# Autodesk Inventor assembly: Prueba_ensamble inercia
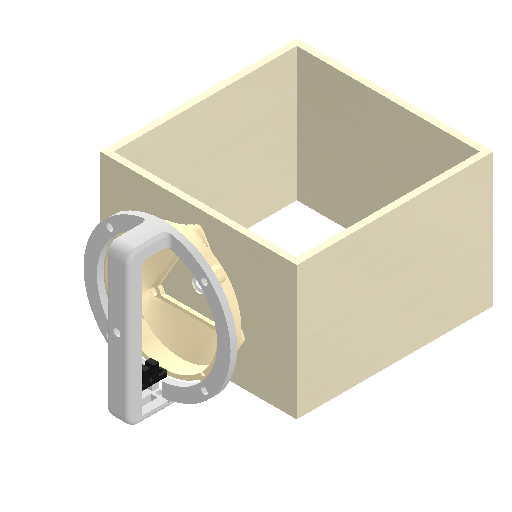
[picture p0: Inventor's stored thumbnail of the model, 512x512]
Saved by Autodesk Inventor 2025.2 (Build 292293000, 293)
## iProperties
Created: 2025-05-05
Part Number: Prueba_ensamble inercia
Document SubType Name: Assembly
Designer: nicoa
Author: nicoa
## Documents named in this file (6)
- C:\Users\nicoa\Documents\FLUSS\Tunel_fluss\Ensamble inercia\Prueba_ensamble inercia.iam
- C:\Users\nicoa\Documents\FLUSS\Tunel_fluss\Ensamble inercia\Seccion_tunel.ipt
- C:\Users\nicoa\Documents\FLUSS\Tunel_fluss\Ensamble inercia\soporte motor.ipt
- C:\Users\nicoa\Documents\FLUSS\Tunel_fluss\Ensamble inercia\Eje_econder.ipt
- C:\Users\nicoa\Documents\FLUSS\Tunel_fluss\Ensamble inercia\Sensor.ipt
- C:\Users\nicoa\Documents\FLUSS\Tunel_fluss\Ensamble inercia\Soporte.ipt
## Components (5 placed, 5 different names)
1. Seccion_tunel:1 — Mate:1, Rotational:1
2. soporte motor:1 — Mate:1, Rotational:1, Mate:2, Mate:3
3. Eje_econder:1
4. Sensor:1
5. Soporte:1 — Mate:2, Mate:3
## Relationships (4: Mate 3, RevoluteJoint 1)
- Mate:1: Seccion_tunel:1 ↔ soporte motor:1
- Rotational:1 [RevoluteJoint]: Seccion_tunel:1 ↔ soporte motor:1
- Mate:2: soporte motor:1 ↔ Soporte:1
- Mate:3: soporte motor:1 ↔ Soporte:1
